# Autodesk Inventor assembly: WheelMotor
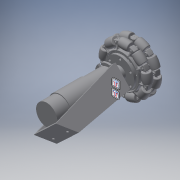
[picture p0: Inventor's stored thumbnail of the model, 180x180]
Saved by Autodesk Inventor 2016 (Build 200138000, 138)
## iProperties
Created: 2015-09-29
Part Number: WheelMotor
Document SubType Name: Assembly
Designer: Mack
Author: Mack
## Documents named in this file (11)
- C:\Users\Mack\code\ballbot\models\WheelMotor.iam
- C:\Users\Mack\code\ballbot\models\217-2584-STEP-20141007\217-2584-002 Rev2.ipt
- C:\Users\Mack\code\ballbot\models\217-2584-STEP-20141007\217-2584-001 Rev1.ipt
- C:\Users\Mack\code\ballbot\models\217-2584-STEP-20141007\217-2584-004 Rev1.ipt
- C:\Users\Mack\code\ballbot\models\217-2584-STEP-20141007\217-2584-003 Rev4.ipt
- C:\Users\Mack\code\ballbot\models\217-2584-STEP-20141007\BEAM-0750.ipt
- C:\Users\Mack\code\ballbot\models\217-2584-STEP-20141007\90116A020_90116A020.ipt
- C:\Users\Mack\code\ballbot\models\217-2584-STEP-20141007\217-2584-005 Rev1 A.ipt
- C:\Users\Mack\code\ballbot\models\8mm-key-hub.ipt
- C:\Users\Mack\code\ballbot\models\motor.ipt
- C:\Users\Mack\code\ballbot\models\MotorMount2.ipt
## Components (102 placed, 102 different names)
1. 217-2584-002 Rev2_1
2. 217-2584-001 Rev1_2
3. 217-2584-001 Rev1_3
4. 217-2584-004 Rev1_4
5. 217-2584-004 Rev1_5
6. 217-2584-004 Rev1_6
7. 217-2584-004 Rev1_7
8. 217-2584-004 Rev1_8
9. 217-2584-004 Rev1_9
10. 217-2584-004 Rev1_10
11. 217-2584-004 Rev1_11
12. 217-2584-004 Rev1_12
13. 217-2584-004 Rev1_13
14. 217-2584-004 Rev1_14
15. 217-2584-004 Rev1_15
16. 217-2584-004 Rev1_16
17. 217-2584-004 Rev1_17
18. 217-2584-004 Rev1_18
19. 217-2584-004 Rev1_19
20. 217-2584-004 Rev1_20
21. 217-2584-004 Rev1_21
22. 217-2584-001 Rev1_22
23. 217-2584-001 Rev1_23
24. 217-2584-001 Rev1_24
25. 217-2584-001 Rev1_25
26. 217-2584-001 Rev1_26
27. 217-2584-001 Rev1_27
28. 217-2584-001 Rev1_28
29. 217-2584-001 Rev1_29
30. 217-2584-001 Rev1_30
31. 217-2584-001 Rev1_31
32. 217-2584-001 Rev1_32
33. 217-2584-001 Rev1_33
34. 217-2584-001 Rev1_34
35. 217-2584-001 Rev1_35
36. 217-2584-001 Rev1_36
37. 217-2584-001 Rev1_37
38. 217-2584-003 Rev4_38
39. 217-2584-003 Rev4_39
40. BEAM-0750_40
41. BEAM-0750_41
42. BEAM-0750_42
43. BEAM-0750_43
44. BEAM-0750_44
45. BEAM-0750_45
46. 90116A020_90116A020_46
47. 90116A020_90116A020_47
48. 90116A020_90116A020_48
49. 90116A020_90116A020_49
50. 90116A020_90116A020_50
51. 90116A020_90116A020_51
52. 90116A020_90116A020_52
53. 90116A020_90116A020_53
54. 90116A020_90116A020_54
55. 90116A020_90116A020_55
56. 90116A020_90116A020_56
57. 90116A020_90116A020_57
58. 90116A020_90116A020_58
59. 90116A020_90116A020_59
60. 90116A020_90116A020_60
61. 90116A020_90116A020_61
62. 90116A020_90116A020_62
63. 90116A020_90116A020_63
64. 217-2584-005 Rev1 A_64
65. 217-2584-005 Rev1 A_65
66. 217-2584-005 Rev1 A_66
67. 217-2584-005 Rev1 A_67
68. 217-2584-005 Rev1 A_68
69. 217-2584-005 Rev1 A_69
70. 217-2584-005 Rev1 A_70
71. 217-2584-005 Rev1 A_71
72. 217-2584-005 Rev1 A_72
73. 217-2584-005 Rev1 A_73
74. 217-2584-005 Rev1 A_74
75. 217-2584-005 Rev1 A_75
76. 217-2584-005 Rev1 A_76
77. 217-2584-005 Rev1 A_77
78. 217-2584-005 Rev1 A_78
79. 217-2584-005 Rev1 A_79
80. 217-2584-005 Rev1 A_80
81. 217-2584-005 Rev1 A_81
82. 217-2584-005 Rev1 A_82
83. 217-2584-005 Rev1 A_83
84. 217-2584-005 Rev1 A_84
85. 217-2584-005 Rev1 A_85
86. 217-2584-005 Rev1 A_86
87. 217-2584-005 Rev1 A_87
88. 217-2584-005 Rev1 A_88
89. 217-2584-005 Rev1 A_89
90. 217-2584-005 Rev1 A_90
91. 217-2584-005 Rev1 A_91
92. 217-2584-005 Rev1 A_92
93. 217-2584-005 Rev1 A_93
94. 217-2584-005 Rev1 A_94
95. 217-2584-005 Rev1 A_95
96. 217-2584-005 Rev1 A_96
97. 217-2584-005 Rev1 A_97
98. 217-2584-005 Rev1 A_98
99. 217-2584-005 Rev1 A_99
100. 8mm-key-hub:1 — Insert:2
101. motor:1 — Insert:2, Insert:5, Insert:6
102. MotorMount2:1 — Insert:5, Insert:6
## Relationships (4: Insert 4)
- [Insert] (3.175 mm): 217-2584-003 Rev4_39 ↔ 8mm-key-hub:1
- Insert:2: 8mm-key-hub:1 ↔ motor:1
- Insert:5: motor:1 ↔ MotorMount2:1
- Insert:6: motor:1 ↔ MotorMount2:1
